# Autodesk Inventor assembly: Bumper Assembly
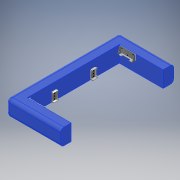
[picture p0: Inventor's stored thumbnail of the model, 180x180]
Saved by Autodesk Inventor 2018 (Build 220112000, 112)
## iProperties
Created: 2020-01-22
Part Number: Bumper Assembly
Document SubType Name: Assembly
Designer: s-2512711
Author: s-2512711
## Documents named in this file (6)
- \\studenthome\students\S-2512711\GitHub\2020CAD\Bumpers\Main Assembly File\Bumper Assembly.iam
- \\studenthome\students\S-2512711\GitHub\2020CAD\Bumpers\Part Files\Bumper Side.ipt
- \\studenthome\students\S-2512711\GitHub\2020CAD\Bumpers\Part Files\am-3961 AM14U4 2019 Front Bumper Bracket.ipt
- \\studenthome\students\S-2512711\GitHub\2020CAD\Bumpers\Part Files\am-3962 AM14U4 2019 Side Bumper Bracket .ipt
- \\studenthome\students\S-2512711\GitHub\2020CAD\Bumpers\Part Files\90294A197_PHILLIPS FLAT HEAD SCREWS FOR WOOD.ipt
- \\studenthome\students\S-2512711\GitHub\2020CAD\Bumpers\Part Files\92001A311_18-8 SS WING NUT.ipt
## Components (23 placed, 5 different names)
1. Bumper Side:1 — Mate:1, Mate:2, Mate:3, Mate:4, Mate:5, Mate:6, Mate:7, Mate:8, Mate:9, Mate:10, Mate:11, Mate:12
2. am-3961 AM14U4 2019 Front Bumper Bracket:1 — Mate:1, Mate:5, Mate:6, Mate:31, Mate:32, Mate:33, Mate:34, Mate:35, Mate:36, Rotation:1, Rotation:2, Rotation:3, Mate:40, Mate:41, Mate:42, Mate:43
3. am-3961 AM14U4 2019 Front Bumper Bracket:2 — Mate:2, Mate:3, Mate:4, Mate:25, Mate:26, Mate:27, Mate:28, Mate:29, Mate:30, Rotation:4, Rotation:5, Rotation:6, Mate:37, Mate:38, Mate:39
4. am-3962 AM14U4 2019 Side Bumper Bracket :1 — Mate:8, Mate:9, Mate:10, Mate:13, Mate:14, Mate:15, Mate:16, Mate:17, Mate:18, Rotation:7, Rotation:8, Rotation:9, Mate:44, Mate:49
5. am-3962 AM14U4 2019 Side Bumper Bracket :2 — Mate:7, Mate:11, Mate:12, Mate:19, Mate:20, Mate:21, Mate:22, Mate:23, Mate:24, Rotation:10, Rotation:11, Rotation:12, Mate:47, Mate:48
6. 90294A197_PHILLIPS FLAT HEAD SCREWS FOR WOOD:1 — Mate:33, Mate:34, Rotation:3
7. 90294A197_PHILLIPS FLAT HEAD SCREWS FOR WOOD:2 — Mate:32, Mate:35, Rotation:2
8. 90294A197_PHILLIPS FLAT HEAD SCREWS FOR WOOD:3 — Mate:31, Mate:36, Rotation:1
9. 90294A197_PHILLIPS FLAT HEAD SCREWS FOR WOOD:4 — Mate:17, Mate:18, Rotation:9
10. 90294A197_PHILLIPS FLAT HEAD SCREWS FOR WOOD:5 — Mate:15, Mate:16, Rotation:8
11. 90294A197_PHILLIPS FLAT HEAD SCREWS FOR WOOD:6 — Mate:13, Mate:14, Rotation:7
12. 90294A197_PHILLIPS FLAT HEAD SCREWS FOR WOOD:7 — Mate:21, Mate:24, Rotation:10
13. 90294A197_PHILLIPS FLAT HEAD SCREWS FOR WOOD:8 — Mate:20, Mate:23, Rotation:11
14. 90294A197_PHILLIPS FLAT HEAD SCREWS FOR WOOD:9 — Mate:19, Mate:22, Rotation:12
15. 90294A197_PHILLIPS FLAT HEAD SCREWS FOR WOOD:10 — Mate:25, Mate:30, Rotation:4
16. 90294A197_PHILLIPS FLAT HEAD SCREWS FOR WOOD:11 — Mate:26, Mate:29, Rotation:5
17. 90294A197_PHILLIPS FLAT HEAD SCREWS FOR WOOD:12 — Mate:27, Mate:28, Rotation:6
18. 92001A311_18-8 SS WING NUT:1 — Mate:44, Mate:49
19. 92001A311_18-8 SS WING NUT:2 — Mate:47, Mate:48
20. 92001A311_18-8 SS WING NUT:3 — Mate:37, Mate:38
21. 92001A311_18-8 SS WING NUT:4 — Mate:39
22. 92001A311_18-8 SS WING NUT:5 — Mate:40, Mate:43
23. 92001A311_18-8 SS WING NUT:6 — Mate:41, Mate:42
## Relationships (59: Mate 47, RelateRotation 12)
- Mate:1: Bumper Side:1 ↔ am-3961 AM14U4 2019 Front Bumper Bracket:1
- Mate:2: Bumper Side:1 ↔ am-3961 AM14U4 2019 Front Bumper Bracket:2
- Mate:3: Bumper Side:1 ↔ am-3961 AM14U4 2019 Front Bumper Bracket:2
- Mate:4: Bumper Side:1 ↔ am-3961 AM14U4 2019 Front Bumper Bracket:2
- Mate:5: Bumper Side:1 ↔ am-3961 AM14U4 2019 Front Bumper Bracket:1
- Mate:6: Bumper Side:1 ↔ am-3961 AM14U4 2019 Front Bumper Bracket:1
- Mate:7: Bumper Side:1 ↔ am-3962 AM14U4 2019 Side Bumper Bracket :2
- Mate:8: Bumper Side:1 ↔ am-3962 AM14U4 2019 Side Bumper Bracket :1
- Mate:9: Bumper Side:1 ↔ am-3962 AM14U4 2019 Side Bumper Bracket :1
- Mate:10: Bumper Side:1 ↔ am-3962 AM14U4 2019 Side Bumper Bracket :1
- Mate:11: Bumper Side:1 ↔ am-3962 AM14U4 2019 Side Bumper Bracket :2
- Mate:12: Bumper Side:1 ↔ am-3962 AM14U4 2019 Side Bumper Bracket :2
- Mate:13: am-3962 AM14U4 2019 Side Bumper Bracket :1 ↔ 90294A197_PHILLIPS FLAT HEAD SCREWS FOR WOOD:6
- Mate:14: am-3962 AM14U4 2019 Side Bumper Bracket :1 ↔ 90294A197_PHILLIPS FLAT HEAD SCREWS FOR WOOD:6
- Mate:15: am-3962 AM14U4 2019 Side Bumper Bracket :1 ↔ 90294A197_PHILLIPS FLAT HEAD SCREWS FOR WOOD:5
- Mate:16: am-3962 AM14U4 2019 Side Bumper Bracket :1 ↔ 90294A197_PHILLIPS FLAT HEAD SCREWS FOR WOOD:5
- Mate:17: am-3962 AM14U4 2019 Side Bumper Bracket :1 ↔ 90294A197_PHILLIPS FLAT HEAD SCREWS FOR WOOD:4
- Mate:18: am-3962 AM14U4 2019 Side Bumper Bracket :1 ↔ 90294A197_PHILLIPS FLAT HEAD SCREWS FOR WOOD:4
- Mate:19: am-3962 AM14U4 2019 Side Bumper Bracket :2 ↔ 90294A197_PHILLIPS FLAT HEAD SCREWS FOR WOOD:9
- Mate:20: am-3962 AM14U4 2019 Side Bumper Bracket :2 ↔ 90294A197_PHILLIPS FLAT HEAD SCREWS FOR WOOD:8
- Mate:21: am-3962 AM14U4 2019 Side Bumper Bracket :2 ↔ 90294A197_PHILLIPS FLAT HEAD SCREWS FOR WOOD:7
- Mate:22: am-3962 AM14U4 2019 Side Bumper Bracket :2 ↔ 90294A197_PHILLIPS FLAT HEAD SCREWS FOR WOOD:9
- Mate:23: am-3962 AM14U4 2019 Side Bumper Bracket :2 ↔ 90294A197_PHILLIPS FLAT HEAD SCREWS FOR WOOD:8
- Mate:24: am-3962 AM14U4 2019 Side Bumper Bracket :2 ↔ 90294A197_PHILLIPS FLAT HEAD SCREWS FOR WOOD:7
- Mate:25: am-3961 AM14U4 2019 Front Bumper Bracket:2 ↔ 90294A197_PHILLIPS FLAT HEAD SCREWS FOR WOOD:10
- Mate:26: am-3961 AM14U4 2019 Front Bumper Bracket:2 ↔ 90294A197_PHILLIPS FLAT HEAD SCREWS FOR WOOD:11
- Mate:27: am-3961 AM14U4 2019 Front Bumper Bracket:2 ↔ 90294A197_PHILLIPS FLAT HEAD SCREWS FOR WOOD:12
- Mate:28: am-3961 AM14U4 2019 Front Bumper Bracket:2 ↔ 90294A197_PHILLIPS FLAT HEAD SCREWS FOR WOOD:12
- Mate:29: am-3961 AM14U4 2019 Front Bumper Bracket:2 ↔ 90294A197_PHILLIPS FLAT HEAD SCREWS FOR WOOD:11
- Mate:30: am-3961 AM14U4 2019 Front Bumper Bracket:2 ↔ 90294A197_PHILLIPS FLAT HEAD SCREWS FOR WOOD:10
- Mate:31: am-3961 AM14U4 2019 Front Bumper Bracket:1 ↔ 90294A197_PHILLIPS FLAT HEAD SCREWS FOR WOOD:3
- Mate:32: am-3961 AM14U4 2019 Front Bumper Bracket:1 ↔ 90294A197_PHILLIPS FLAT HEAD SCREWS FOR WOOD:2
- Mate:33: am-3961 AM14U4 2019 Front Bumper Bracket:1 ↔ 90294A197_PHILLIPS FLAT HEAD SCREWS FOR WOOD:1
- Mate:34: am-3961 AM14U4 2019 Front Bumper Bracket:1 ↔ 90294A197_PHILLIPS FLAT HEAD SCREWS FOR WOOD:1
- Mate:35: am-3961 AM14U4 2019 Front Bumper Bracket:1 ↔ 90294A197_PHILLIPS FLAT HEAD SCREWS FOR WOOD:2
- Mate:36: am-3961 AM14U4 2019 Front Bumper Bracket:1 ↔ 90294A197_PHILLIPS FLAT HEAD SCREWS FOR WOOD:3
- Rotation:1 [RelateRotation] (1 ul): am-3961 AM14U4 2019 Front Bumper Bracket:1 ↔ 90294A197_PHILLIPS FLAT HEAD SCREWS FOR WOOD:3
- Rotation:2 [RelateRotation] (1 ul): am-3961 AM14U4 2019 Front Bumper Bracket:1 ↔ 90294A197_PHILLIPS FLAT HEAD SCREWS FOR WOOD:2
- Rotation:3 [RelateRotation] (1 ul): am-3961 AM14U4 2019 Front Bumper Bracket:1 ↔ 90294A197_PHILLIPS FLAT HEAD SCREWS FOR WOOD:1
- Rotation:4 [RelateRotation] (1 ul): am-3961 AM14U4 2019 Front Bumper Bracket:2 ↔ 90294A197_PHILLIPS FLAT HEAD SCREWS FOR WOOD:10
- Rotation:5 [RelateRotation] (1 ul): am-3961 AM14U4 2019 Front Bumper Bracket:2 ↔ 90294A197_PHILLIPS FLAT HEAD SCREWS FOR WOOD:11
- Rotation:6 [RelateRotation] (1 ul): am-3961 AM14U4 2019 Front Bumper Bracket:2 ↔ 90294A197_PHILLIPS FLAT HEAD SCREWS FOR WOOD:12
- Rotation:7 [RelateRotation] (1 ul): am-3962 AM14U4 2019 Side Bumper Bracket :1 ↔ 90294A197_PHILLIPS FLAT HEAD SCREWS FOR WOOD:6
- Rotation:8 [RelateRotation] (1 ul): am-3962 AM14U4 2019 Side Bumper Bracket :1 ↔ 90294A197_PHILLIPS FLAT HEAD SCREWS FOR WOOD:5
- Rotation:9 [RelateRotation] (1 ul): am-3962 AM14U4 2019 Side Bumper Bracket :1 ↔ 90294A197_PHILLIPS FLAT HEAD SCREWS FOR WOOD:4
- Rotation:10 [RelateRotation] (1 ul): am-3962 AM14U4 2019 Side Bumper Bracket :2 ↔ 90294A197_PHILLIPS FLAT HEAD SCREWS FOR WOOD:7
- Rotation:11 [RelateRotation] (1 ul): am-3962 AM14U4 2019 Side Bumper Bracket :2 ↔ 90294A197_PHILLIPS FLAT HEAD SCREWS FOR WOOD:8
- Rotation:12 [RelateRotation] (1 ul): am-3962 AM14U4 2019 Side Bumper Bracket :2 ↔ 90294A197_PHILLIPS FLAT HEAD SCREWS FOR WOOD:9
- Mate:37: am-3961 AM14U4 2019 Front Bumper Bracket:2 ↔ 92001A311_18-8 SS WING NUT:3
- Mate:38: am-3961 AM14U4 2019 Front Bumper Bracket:2 ↔ 92001A311_18-8 SS WING NUT:3
- Mate:39: am-3961 AM14U4 2019 Front Bumper Bracket:2 ↔ 92001A311_18-8 SS WING NUT:4
- Mate:40: am-3961 AM14U4 2019 Front Bumper Bracket:1 ↔ 92001A311_18-8 SS WING NUT:5
- Mate:41: am-3961 AM14U4 2019 Front Bumper Bracket:1 ↔ 92001A311_18-8 SS WING NUT:6
- Mate:42: am-3961 AM14U4 2019 Front Bumper Bracket:1 ↔ 92001A311_18-8 SS WING NUT:6
- Mate:43: am-3961 AM14U4 2019 Front Bumper Bracket:1 ↔ 92001A311_18-8 SS WING NUT:5
- Mate:44 (3.175 mm): am-3962 AM14U4 2019 Side Bumper Bracket :1 ↔ 92001A311_18-8 SS WING NUT:1
- Mate:47 (3.175 mm): am-3962 AM14U4 2019 Side Bumper Bracket :2 ↔ 92001A311_18-8 SS WING NUT:2
- Mate:48: am-3962 AM14U4 2019 Side Bumper Bracket :2 ↔ 92001A311_18-8 SS WING NUT:2
- Mate:49: am-3962 AM14U4 2019 Side Bumper Bracket :1 ↔ 92001A311_18-8 SS WING NUT:1
